# Autodesk Inventor assembly: Connessione A
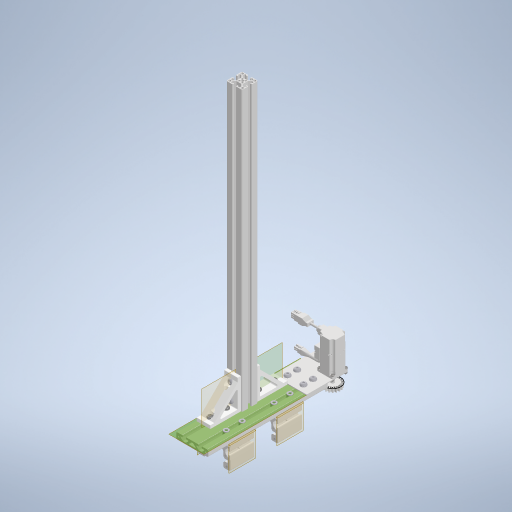
[picture p0: Inventor's stored thumbnail of the model, 512x512]
Saved by Autodesk Inventor 2023 (Build 270158000, 158)
## iProperties
Created: 2022-08-25
Part Number: Connessione A
Document SubType Name: Assembly
Designer: matte
Author: matte
## Documents named in this file (5)
- C:\Users\matte\Documents\GitHub\MDM-CyberOrto-CAD\Esplosi\Connessione A.iam
- C:\Users\matte\Documents\GitHub\MDM-CyberOrto-CAD\Pezzi singoli\Supporto SX.ipt
- C:\Users\matte\Documents\GitHub\MDM-CyberOrto-CAD\Guida a terra.iam
- C:\Users\matte\Documents\GitHub\MDM-CyberOrto-CAD\Rack_Pinion\Motor_assembly.iam
- C:\Users\matte\Documents\GitHub\MDM-CyberOrto-CAD\Parker components\02-Fasteners\10-Standard T-Nuts\20-050.ipt
## Components (5 placed, 4 different names)
1. Supporto SX:1 — Coincidente:9, Coincidente:10
2. Guida a terra:1 [sub-assembly] — Coincidente:5, Coincidente:6, Coincidente:7, Coincidente:8
3. Motor_assembly:1 [sub-assembly]
4. 20-050:1 — Coincidente:5, Coincidente:6, Coincidente:10
5. 20-050:2 — Coincidente:7, Coincidente:8, Coincidente:9
## Relationships (12: Mate 10, Flush 2)
- [Mate]: Supporto SX:1 ↔ Guida a terra:1
- [Mate]: Supporto SX:1 ↔ Guida a terra:1
- [Mate]: Supporto SX:1 ↔ Guida a terra:1
- [Mate]: Guida a terra:1 ↔ Motor_assembly:1
- [Flush]: Guida a terra:1 ↔ Motor_assembly:1
- [Flush] (10 mm): Guida a terra:1 ↔ Motor_assembly:1
- Coincidente:5 [Mate]: Guida a terra:1 ↔ 20-050:1
- Coincidente:6 [Mate]: Guida a terra:1 ↔ 20-050:1
- Coincidente:7 [Mate]: Guida a terra:1 ↔ 20-050:2
- Coincidente:8 [Mate]: Guida a terra:1 ↔ 20-050:2
- Coincidente:9 [Mate]: Supporto SX:1 ↔ 20-050:2
- Coincidente:10 [Mate]: Supporto SX:1 ↔ 20-050:1
